# Autodesk Inventor assembly: Montagem da fixação do sensor de temperatura
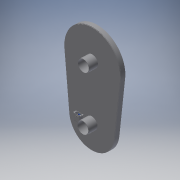
[picture p0: Inventor's stored thumbnail of the model, 180x180]
Saved by Autodesk Inventor 2019 (Build 230136000, 136)
## iProperties
Created: 2020-05-31
Part Number: Montagem da fixação do sensor de temperatura
Material: Genérico
Document SubType Name: Assembly
Designer: Público
Author: Público
## Documents named in this file (6)
- G:\Meu Drive\Projetos\Projeto 2020 2021\Eletrônica 2020-2021\Projeção mecânica\Fixação do sensor de temperatura\Montagem da fixação do sensor de temperatura.iam
- G:\Meu Drive\Projetos\Projeto 2020 2021\Eletrônica 2020-2021\Projeção mecânica\Fixação do sensor de temperatura\Tampa capa CVT.ipt
- G:\Meu Drive\Projetos\Projeto 2020 2021\Eletrônica 2020-2021\Projeção mecânica\Fixação do sensor de temperatura\Sensor de temperatura.ipt
- G:\Meu Drive\Projetos\Projeto 2020 2021\Eletrônica 2020-2021\Projeção mecânica\Fixação do sensor de temperatura\Caixa do sensor de temperatura.ipt
- C:\Users\Arlison\Documents\Inventor\Content Center Files\R2019\pt-BR\GB 5784-86\Bolt GB 5784-86-M3 x 20.ipt
- C:\Users\Arlison\Documents\Inventor\Content Center Files\R2019\pt-BR\ANSI B18.2.4.2M\ANSI B18.2.4.2M - M3x0,5 - 5,5.ipt
## Components (7 placed, 5 different names)
1. Tampa capa CVT:1 — Coincidência:2, Inserir:1, Inserir:2
2. Sensor de temperatura:1 — Coincidência:1
3. Caixa do sensor de temperatura:1 — Coincidência:1, Coincidência:2
4. Bolt GB/T 5784-1986 M3x20:1
5. Bolt GB/T 5784-1986 M3x20:2
6. ANSI B18.2.4.2M M3x0,5:1 — Inserir:1
7. ANSI B18.2.4.2M M3x0,5:2 — Inserir:2
## Relationships (4: Mate 2, Insert 2)
- Coincidência:1 [Mate]: Sensor de temperatura:1 ↔ Caixa do sensor de temperatura:1
- Coincidência:2 [Mate]: Tampa capa CVT:1 ↔ Caixa do sensor de temperatura:1
- Inserir:1: Tampa capa CVT:1 ↔ ANSI B18.2.4.2M M3x0,5:1
- Inserir:2: Tampa capa CVT:1 ↔ ANSI B18.2.4.2M M3x0,5:2
